# Autodesk Inventor assembly: foot_ass
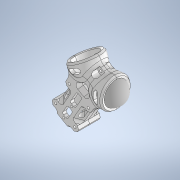
[picture p0: Inventor's stored thumbnail of the model, 180x180]
Saved by Autodesk Inventor 2020 (Build 240168000, 168)
## iProperties
Created: 2020-10-06
Part Number: foot_ass
Document SubType Name: Assembly
Designer: Shuang Peng
Author: Shuang Peng
## Documents named in this file (3)
- D:\projects-3\biped_gen1\hardware\foot_ass.iam
- D:\projects-3\biped_gen1\hardware\legend_40mm.ipt
- D:\projects-3\biped_gen1\hardware\foot_1.ipt
## Components (3 placed, 2 different names)
1. legend_40mm:1 — Tangent:1
2. foot_1:1 — Tangent:1, Insert:1, Insert:2
3. foot_1:2 — Insert:1, Insert:2
## Relationships (3: Insert 2, Tangent 1)
- Tangent:1: legend_40mm:1 ↔ foot_1:1
- Insert:1: foot_1:1 ↔ foot_1:2
- Insert:2: foot_1:1 ↔ foot_1:2
